# Autodesk Inventor assembly: ASM_Tool_Tip_Rev_seperate
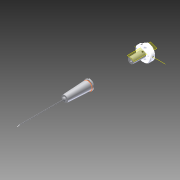
[picture p0: Inventor's stored thumbnail of the model, 180x180]
Saved by Autodesk Inventor 2011 SP2 (Build 150309200, 309)
## iProperties
Created: 2011-08-18
Part Number: ASM_Tool_Tip_Rev_seperate
Document SubType Name: Assembly
Designer: sungwook
Author: sungwook
## Documents named in this file (5)
- C:\Users\sungwook\Documents\Inventor\Micron22_top_adj_02082013\Parts\Tool\ASM_Tool_Tip_Rev_seperate.iam
- C:\Users\sungwook\Documents\Inventor\Micron22_top_adj_02082013\Parts\Tool\Tool Mount_Rev.ipt
- C:\Users\sungwook\Documents\Inventor\Micron22_top_adj_02082013\Parts\Tool\Tool_Mount_Luer_Adapter.ipt
- C:\Users\sungwook\Documents\Inventor\Content Center Files\R2011\en-US\ANSI B18.3(18)\ANSI B18.3 - 0-80 UNF - 0.13(28).ipt
- C:\Users\sungwook\Documents\Inventor\Micron22_top_adj_02082013\Parts\Tool\Needle_Asm.iam
## Components (5 placed, 4 different names)
1. Tool Mount_Rev:1 — Mate:1, Mate:2, Mate:5, Mate:6, Mate:8, Angle:1
2. Tool_Mount_Luer_Adapter:1 — Mate:1, Mate:2, Mate:7
3. Needle_Asm:1 [sub-assembly] — Mate:7, Mate:8, Angle:1
4. Type A - Hexagon Socket Set Screw - Cup Point - Inch 0-80 UNF x 0.13:1 — Mate:5, Mate:6
5. Type A - Hexagon Socket Set Screw - Cup Point - Inch 0-80 UNF x 0.13:2
## Component patterns: (2 elements, first: Type A - Hexagon Socket Set Screw - Cup Point - Inch 0-80 UNF x 0.13:1)
## Relationships (7: Mate 6, Angle 1)
- Mate:1: Tool Mount_Rev:1 ↔ Tool_Mount_Luer_Adapter:1
- Mate:2: Tool Mount_Rev:1 ↔ Tool_Mount_Luer_Adapter:1
- Mate:5: Tool Mount_Rev:1 ↔ Type A - Hexagon Socket Set Screw - Cup Point - Inch 0-80 UNF x 0.13:1
- Mate:6 (1.2333 mm): Tool Mount_Rev:1 ↔ Type A - Hexagon Socket Set Screw - Cup Point - Inch 0-80 UNF x 0.13:1
- Mate:7: Tool_Mount_Luer_Adapter:1 ↔ Needle_Asm:1
- Mate:8 (2.5 mm): Tool Mount_Rev:1 ↔ Needle_Asm:1
- Angle:1 (60 deg): Tool Mount_Rev:1 ↔ Needle_Asm:1
